# Autodesk Inventor assembly: CLIM_000_ClimbAssembly
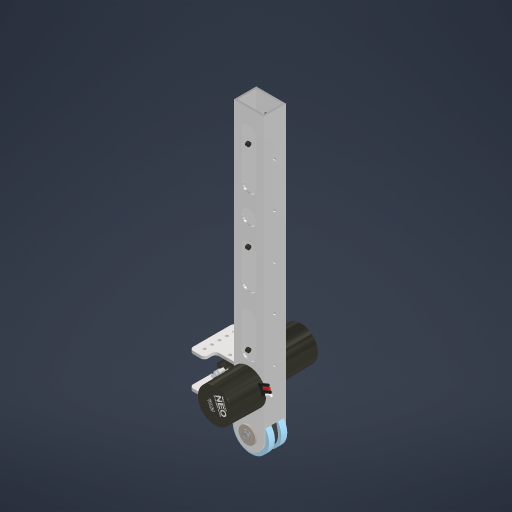
[picture p0: Inventor's stored thumbnail of the model, 512x512]
Saved by Autodesk Inventor 2024.2 (Build 282272000, 272)
## iProperties
Created: 2024-08-08
Part Number: CLIM_000_ClimbAssembly
Document SubType Name: Assembly
Designer: Bryan
Mass: 1242 g
Surface Area: 2302.8 cm^2
Volume: 436.098 cm^3
Density: 2.84798 g/cm^3
Author: Bryan
## Documents named in this file (15)
- C:\Users\bobsb\OneDrive\Documents\GitHub\1622-2024-Summer-CAD-A-Thon\Climb\CLIM_000_ClimbAssembly.iam
- C:\Users\bobsb\OneDrive\Documents\GitHub\1622-2024-Summer-CAD-A-Thon\Climb\CLIM_002_ClimbPole.ipt
- C:\Users\bobsb\OneDrive\Documents\GitHub\1622-2024-Summer-CAD-A-Thon\Climb\CLIM_001_ClimbRack.ipt
- C:\Users\bobsb\OneDrive\Documents\GitHub\1622-2024-Summer-CAD-A-Thon\COTS Library\Motion\Bearings\COTS_WCP-0781_0.5ODCircularFlangedBearing.ipt
- C:\Users\bobsb\OneDrive\Documents\GitHub\1622-2024-Summer-CAD-A-Thon\Climb\CLIM_003_RollerPulley.ipt
- C:\Users\bobsb\OneDrive\Documents\GitHub\1622-2024-Summer-CAD-A-Thon\COTS Library\Motors\COTS_REV-21-1650-V1.1_Neo1.1.ipt
- C:\Users\bobsb\OneDrive\Documents\GitHub\1622-2024-Summer-CAD-A-Thon\COTS Library\Fasteners\Bolts\Socket-Head\10-32\COTS_91251A340_Black-Oxide Alloy Steel Socket Head Screw.ipt
- C:\Users\bobsb\OneDrive\Documents\GitHub\1622-2024-Summer-CAD-A-Thon\COTS Library\Motion\Pulleys\HTD5M\10mm Wide\COTW_HTD5M10mm12T_WCP-0076.ipt
- C:\Users\bobsb\OneDrive\Documents\GitHub\1622-2024-Summer-CAD-A-Thon\Climb\CLIM_004_RollerBelt.ipt
- C:\Users\bobsb\OneDrive\Documents\GitHub\1622-2024-Summer-CAD-A-Thon\Climb\CLIM_005_Shaft.ipt
- C:\Users\bobsb\OneDrive\Documents\GitHub\1622-2024-Summer-CAD-A-Thon\COTS Library\Fasteners\Bolts\Button-Head\0.25-20\COTS_0.25-20_ButtonHead_0.5inlong_StainlessSteel_92949A537.ipt
- C:\Users\bobsb\OneDrive\Documents\GitHub\1622-2024-Summer-CAD-A-Thon\COTS Library\Fasteners\Washers\COTS_90107A029_316 Stainless Steel Washer.ipt
- C:\Users\bobsb\OneDrive\Documents\GitHub\1622-2024-Summer-CAD-A-Thon\COTS Library\Fasteners\Bolts\Socket-Head\8-32\COTS_3-8in_91251A192_Black-Oxide Alloy Steel Socket Head Screw.ipt
- C:\Users\bobsb\OneDrive\Documents\GitHub\1622-2024-Summer-CAD-A-Thon\Drive Base\DVBS_003_MAXTube26in.ipt
- C:\Users\bobsb\OneDrive\Documents\GitHub\1622-2024-Summer-CAD-A-Thon\Climb\CLIM_008_ClimbBox.iam
## Components (24 placed, 14 different names)
1. CLIM_002_ClimbPole:1 — Mate:2, Mate:3, Mate:4, Mate:5, Mate:6, Mate:7, Mate:10, Mate:11, Mate:12, Mate:13, Mate:14, Mate:15, Mate:16, Mate:17, Mate:32
2. CLIM_001_ClimbRack:1 — Mate:2, Mate:3, Mate:31, Mate:35, Mate:38
3. COTS_WCP-0781_0.5ODCircularFlangedBearing:1 — Mate:4, Mate:5, Mate:8, Mate:9, Mate:25
4. COTS_WCP-0781_0.5ODCircularFlangedBearing:2 — Mate:6, Mate:7, Mate:22, Flush:5, Mate:23, Mate:24
5. CLIM_003_RollerPulley:1 — Mate:8, Mate:9, Flush:4, Mate:19, Mate:21, Tangent:1
6. COTS_REV-21-1650-V1.1_Neo1.1:1 — Mate:10, Mate:11, Mate:12, Mate:18
7. COTS_91251A340_Black-Oxide Alloy Steel Socket Head Screw:1 — Mate:13, Flush:1, Flush:2
8. COTS_91251A340_Black-Oxide Alloy Steel Socket Head Screw:2 — Mate:15, Flush:3
9. COTS_91251A340_Black-Oxide Alloy Steel Socket Head Screw:3 — Mate:16, Flush:2, Flush:3
10. COTS_91251A340_Black-Oxide Alloy Steel Socket Head Screw:4 — Mate:14, Mate:17, Flush:1
11. COTW_HTD5M10mm12T_WCP-0076:1 — Mate:18, Flush:4, Mate:20
12. CLIM_004_RollerBelt:1 — Mate:19, Mate:20, Mate:21
13. CLIM_005_Shaft:1 — Mate:22, Flush:5, Mate:26, Mate:27, Mate:28
14. COTS_0.25-20_ButtonHead_0.5inlong_StainlessSteel_92949A537:1 — Mate:27, Mate:30
15. COTS_0.25-20_ButtonHead_0.5inlong_StainlessSteel_92949A537:2 — Mate:28, Mate:29
16. COTS_90107A029_316 Stainless Steel Washer:1 — Mate:23, Mate:24, Mate:29
17. COTS_90107A029_316 Stainless Steel Washer:2 — Mate:25, Mate:26, Mate:30
18. DVBS_003_MAXTube26in:1 — Mate:33, Mate:35, Flush:6, Mate:39, Mate:40
19. CLIM_008_ClimbBox:1 [sub-assembly] — Mate:38, Flush:6, Mate:39, Mate:40
20. COTS_3-8in_91251A192_Black-Oxide Alloy Steel Socket Head Screw:2 — Mate:31, Mate:32
21. COTS_3-8in_91251A192_Black-Oxide Alloy Steel Socket Head Screw:3
22. COTS_3-8in_91251A192_Black-Oxide Alloy Steel Socket Head Screw:4
23. COTS_3-8in_91251A192_Black-Oxide Alloy Steel Socket Head Screw:5
24. COTS_3-8in_91251A192_Black-Oxide Alloy Steel Socket Head Screw:6
## Component patterns: (5 elements, first: COTS_3-8in_91251A192_Black-Oxide Alloy Steel Socket Head Screw:2)
## Relationships (43: Mate 36, Flush 6, Tangent 1)
- Mate:2: CLIM_002_ClimbPole:1 ↔ CLIM_001_ClimbRack:1
- Mate:3: CLIM_002_ClimbPole:1 ↔ CLIM_001_ClimbRack:1
- Mate:4: CLIM_002_ClimbPole:1 ↔ COTS_WCP-0781_0.5ODCircularFlangedBearing:1
- Mate:5: CLIM_002_ClimbPole:1 ↔ COTS_WCP-0781_0.5ODCircularFlangedBearing:1
- Mate:6: CLIM_002_ClimbPole:1 ↔ COTS_WCP-0781_0.5ODCircularFlangedBearing:2
- Mate:7: CLIM_002_ClimbPole:1 ↔ COTS_WCP-0781_0.5ODCircularFlangedBearing:2
- Mate:8: COTS_WCP-0781_0.5ODCircularFlangedBearing:1 ↔ CLIM_003_RollerPulley:1
- Mate:9: COTS_WCP-0781_0.5ODCircularFlangedBearing:1 ↔ CLIM_003_RollerPulley:1
- Mate:10: CLIM_002_ClimbPole:1 ↔ COTS_REV-21-1650-V1.1_Neo1.1:1
- Mate:11: CLIM_002_ClimbPole:1 ↔ COTS_REV-21-1650-V1.1_Neo1.1:1
- Mate:12: CLIM_002_ClimbPole:1 ↔ COTS_REV-21-1650-V1.1_Neo1.1:1
- Mate:13: CLIM_002_ClimbPole:1 ↔ COTS_91251A340_Black-Oxide Alloy Steel Socket Head Screw:1
- Mate:14: CLIM_002_ClimbPole:1 ↔ COTS_91251A340_Black-Oxide Alloy Steel Socket Head Screw:4
- Mate:15: CLIM_002_ClimbPole:1 ↔ COTS_91251A340_Black-Oxide Alloy Steel Socket Head Screw:2
- Mate:16: CLIM_002_ClimbPole:1 ↔ COTS_91251A340_Black-Oxide Alloy Steel Socket Head Screw:3
- Mate:17: CLIM_002_ClimbPole:1 ↔ COTS_91251A340_Black-Oxide Alloy Steel Socket Head Screw:4
- Flush:1: COTS_91251A340_Black-Oxide Alloy Steel Socket Head Screw:1 ↔ COTS_91251A340_Black-Oxide Alloy Steel Socket Head Screw:4
- Flush:2: COTS_91251A340_Black-Oxide Alloy Steel Socket Head Screw:1 ↔ COTS_91251A340_Black-Oxide Alloy Steel Socket Head Screw:3
- Flush:3: COTS_91251A340_Black-Oxide Alloy Steel Socket Head Screw:2 ↔ COTS_91251A340_Black-Oxide Alloy Steel Socket Head Screw:3
- Mate:18: COTS_REV-21-1650-V1.1_Neo1.1:1 ↔ COTW_HTD5M10mm12T_WCP-0076:1
- Flush:4: CLIM_003_RollerPulley:1 ↔ COTW_HTD5M10mm12T_WCP-0076:1
- Mate:19: CLIM_003_RollerPulley:1 ↔ CLIM_004_RollerBelt:1
- Mate:20: COTW_HTD5M10mm12T_WCP-0076:1 ↔ CLIM_004_RollerBelt:1
- Mate:21: CLIM_003_RollerPulley:1 ↔ CLIM_004_RollerBelt:1
- Mate:22: COTS_WCP-0781_0.5ODCircularFlangedBearing:2 ↔ CLIM_005_Shaft:1
- Flush:5: COTS_WCP-0781_0.5ODCircularFlangedBearing:2 ↔ CLIM_005_Shaft:1
- Mate:23: COTS_WCP-0781_0.5ODCircularFlangedBearing:2 ↔ COTS_90107A029_316 Stainless Steel Washer:1
- Mate:24: COTS_WCP-0781_0.5ODCircularFlangedBearing:2 ↔ COTS_90107A029_316 Stainless Steel Washer:1
- Mate:25: COTS_WCP-0781_0.5ODCircularFlangedBearing:1 ↔ COTS_90107A029_316 Stainless Steel Washer:2
- Mate:26: CLIM_005_Shaft:1 ↔ COTS_90107A029_316 Stainless Steel Washer:2
- Mate:27: CLIM_005_Shaft:1 ↔ COTS_0.25-20_ButtonHead_0.5inlong_StainlessSteel_92949A537:1
- Mate:28: CLIM_005_Shaft:1 ↔ COTS_0.25-20_ButtonHead_0.5inlong_StainlessSteel_92949A537:2
- Mate:29: COTS_0.25-20_ButtonHead_0.5inlong_StainlessSteel_92949A537:2 ↔ COTS_90107A029_316 Stainless Steel Washer:1
- Mate:30: COTS_0.25-20_ButtonHead_0.5inlong_StainlessSteel_92949A537:1 ↔ COTS_90107A029_316 Stainless Steel Washer:2
- Mate:31: CLIM_001_ClimbRack:1 ↔ COTS_3-8in_91251A192_Black-Oxide Alloy Steel Socket Head Screw:2
- Mate:32: CLIM_002_ClimbPole:1 ↔ COTS_3-8in_91251A192_Black-Oxide Alloy Steel Socket Head Screw:2
- Mate:33 (38.1 mm): DVBS_003_MAXTube26in:1
- Tangent:1: CLIM_003_RollerPulley:1
- Mate:35 (3.175 mm): CLIM_001_ClimbRack:1 ↔ DVBS_003_MAXTube26in:1
- Mate:38 (23.495 mm): CLIM_001_ClimbRack:1 ↔ CLIM_008_ClimbBox:1
- Flush:6: DVBS_003_MAXTube26in:1 ↔ CLIM_008_ClimbBox:1
- Mate:39: DVBS_003_MAXTube26in:1 ↔ CLIM_008_ClimbBox:1
- Mate:40: DVBS_003_MAXTube26in:1 ↔ CLIM_008_ClimbBox:1
